# Autodesk Inventor assembly: Assembly_Opentrons_Autofocus_v1
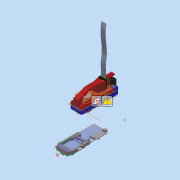
[picture p0: Inventor's stored thumbnail of the model, 180x180]
Saved by Autodesk Inventor 2019.4 (Build 234330000, 330)
## iProperties
Created: 2020-10-23
Part Number: Assembly_Opentrons_Autofocus_v1
Document SubType Name: Assembly
Designer: diederichbenedict
Author: diederichbenedict
## Documents named in this file (17)
- C:\Users\diederichbenedict\Dropbox\Dokumente\Promotion\PROJECTS\OPENTRONS\INVENTOR\Assembly_Opentrons_Autofocus_v1.iam
- C:\Users\diederichbenedict\Dropbox\Dokumente\Promotion\PROJECTS\OPENTRONS\INVENTOR\00_RasPi_Camera.ipt
- C:\Users\diederichbenedict\Dropbox\Dokumente\Promotion\PROJECTS\OPENTRONS\INVENTOR\00_IGUS_Drylin_RJ4JP-01-06.ipt
- C:\Users\diederichbenedict\Dropbox\Dokumente\Promotion\PROJECTS\OPENTRONS\INVENTOR\00_spindel_slide.ipt
- C:\Users\diederichbenedict\Dropbox\Dokumente\Promotion\PROJECTS\OPENTRONS\INVENTOR\00_JF-0530B-solenoid.ipt
- C:\Users\diederichbenedict\Dropbox\Dokumente\Promotion\PROJECTS\OPENTRONS\INVENTOR\00_objectivelens_10x.ipt
- C:\Users\diederichbenedict\Dropbox\Dokumente\Promotion\PROJECTS\OPENTRONS\INVENTOR\01_Slide_camera_x_v1.ipt
- C:\Users\diederichbenedict\Dropbox\Dokumente\Promotion\PROJECTS\OPENTRONS\INVENTOR\00_opticalpath.ipt
- C:\Users\diederichbenedict\Dropbox\Dokumente\Promotion\PROJECTS\OPENTRONS\INVENTOR\07_OPENTRONS_Autofocus_objectivemount_v0.ipt
- C:\Users\diederichbenedict\Dropbox\Dokumente\Promotion\PROJECTS\OPENTRONS\INVENTOR\00_COMAR_Mirror_10mm.ipt
- C:\Users\diederichbenedict\Dropbox\Dokumente\Promotion\PROJECTS\OPENTRONS\INVENTOR\08_Opentrons_Autofocus_flexurebaering.ipt
- C:\Users\diederichbenedict\Dropbox\Dokumente\Promotion\PROJECTS\OPENTRONS\INVENTOR\09_Opentrons_Autofocus_LED_Module.ipt
- C:\Users\diederichbenedict\Dropbox\Dokumente\Promotion\PROJECTS\OPENTRONS\INVENTOR\Assembly_Opentrons_Autofocus_Measure_v0.iam
- C:\Users\diederichbenedict\Dropbox\Dokumente\Promotion\PROJECTS\OPENTRONS\INVENTOR\00_ESP32_Camera_only.ipt
- C:\Users\diederichbenedict\Dropbox\Dokumente\Promotion\PROJECTS\OPENTRONS\INVENTOR\00_Beampath_Autofocus _2.ipt
- C:\Users\diederichbenedict\Dropbox\Dokumente\Promotion\PROJECTS\OPENTRONS\INVENTOR\00_IR_Laserdiode.ipt
- C:\Users\diederichbenedict\Dropbox\Dokumente\Promotion\PROJECTS\OPENTRONS\INVENTOR\13_Opentrons_Autofocus_Objectivering_Laser_Cam.ipt
## Components (16 placed, 16 different names)
1. 00_IGUS_Drylin_RJ4JP-01-06:1
2. 00_spindel_slide:1 — Insert:5
3. 01_Slide_camera_x_v1:1 — Insert:5, Mate:1, Mate:2, Flush:4, Angle:2, Flush:5, Flush:6, Angle:3, Angle:4, Flush:8, Flush:11
4. 00_JF-0530B-solenoid:1 — Insert:9, Angle:3
5. 00_objectivelens_10x:1 — Mate:1, Mate:2, Flush:2, Insert:10
6. 00_opticalpath:1 — Flush:4, Insert:7, Insert:8, Flush:7, Flush:9
7. 07_OPENTRONS_Autofocus_objectivemount_v0:1 — Flush:2
8. 00_COMAR_Mirror_10mm:1 — Insert:7
9. 00_RasPi_Camera:1 — Insert:8, Angle:2
10. 08_Opentrons_Autofocus_flexurebaering:1 — Flush:5, Flush:6, Insert:9, Flush:7
11. Assembly_Opentrons_Autofocus_Measure_v0:1 [sub-assembly]
12. 00_ESP32_Camera_only:1 — Mate:4, Mate:5, Angle:5
13. 09_Opentrons_Autofocus_LED_Module:1
14. 00_Beampath_Autofocus _2:1 — Insert:10, Mate:3, Mate:4, Angle:4
15. 00_IR_Laserdiode:1 — Mate:3, Flush:10
16. 13_Opentrons_Autofocus_Objectivering_Laser_Cam:1 — Flush:8, Flush:9, Flush:10, Flush:11, Mate:5, Angle:5
## Relationships (23: Flush 9, Insert 5, Mate 5, Angle 4)
- Insert:5: 00_spindel_slide:1 ↔ 01_Slide_camera_x_v1:1
- Mate:1: 01_Slide_camera_x_v1:1 ↔ 00_objectivelens_10x:1
- Mate:2 (17 mm): 01_Slide_camera_x_v1:1 ↔ 00_objectivelens_10x:1
- Flush:2: 00_objectivelens_10x:1 ↔ 07_OPENTRONS_Autofocus_objectivemount_v0:1
- Flush:4: 01_Slide_camera_x_v1:1 ↔ 00_opticalpath:1
- Insert:7: 00_opticalpath:1 ↔ 00_COMAR_Mirror_10mm:1
- Insert:8: 00_opticalpath:1 ↔ 00_RasPi_Camera:1
- Angle:2 (90 deg): 01_Slide_camera_x_v1:1 ↔ 00_RasPi_Camera:1
- Flush:5: 01_Slide_camera_x_v1:1 ↔ 08_Opentrons_Autofocus_flexurebaering:1
- Flush:6: 01_Slide_camera_x_v1:1 ↔ 08_Opentrons_Autofocus_flexurebaering:1
- Insert:9 (-4 mm): 00_JF-0530B-solenoid:1 ↔ 08_Opentrons_Autofocus_flexurebaering:1
- Angle:3 (90 deg): 01_Slide_camera_x_v1:1 ↔ 00_JF-0530B-solenoid:1
- Flush:7: 00_opticalpath:1 ↔ 08_Opentrons_Autofocus_flexurebaering:1
- Insert:10 (-2 mm): 00_objectivelens_10x:1 ↔ 00_Beampath_Autofocus _2:1
- Mate:3: 00_Beampath_Autofocus _2:1 ↔ 00_IR_Laserdiode:1
- Mate:4: 00_ESP32_Camera_only:1 ↔ 00_Beampath_Autofocus _2:1
- Angle:4 (145 deg): 01_Slide_camera_x_v1:1 ↔ 00_Beampath_Autofocus _2:1
- Flush:8: 01_Slide_camera_x_v1:1 ↔ 13_Opentrons_Autofocus_Objectivering_Laser_Cam:1
- Flush:9: 00_opticalpath:1 ↔ 13_Opentrons_Autofocus_Objectivering_Laser_Cam:1
- Flush:10: 00_IR_Laserdiode:1 ↔ 13_Opentrons_Autofocus_Objectivering_Laser_Cam:1
- Flush:11: 01_Slide_camera_x_v1:1 ↔ 13_Opentrons_Autofocus_Objectivering_Laser_Cam:1
- Mate:5: 00_ESP32_Camera_only:1 ↔ 13_Opentrons_Autofocus_Objectivering_Laser_Cam:1
- Angle:5 (0 deg): 00_ESP32_Camera_only:1 ↔ 13_Opentrons_Autofocus_Objectivering_Laser_Cam:1
